# Autodesk Inventor assembly: head
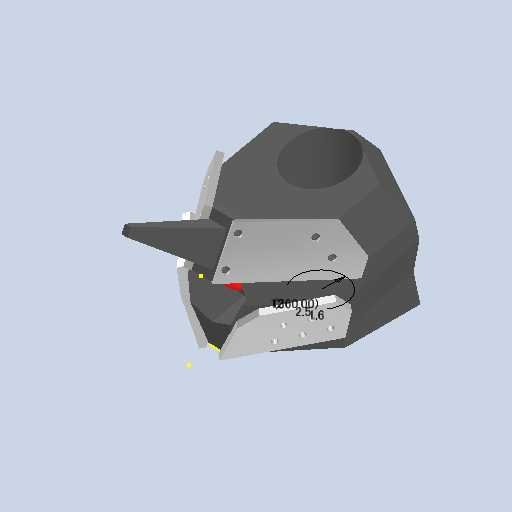
[picture p0: Inventor's stored thumbnail of the model, 512x512]
Saved by Autodesk Inventor 2024.1 (Build 281209000, 209)
## iProperties
Created: 2024-02-25
Part Number: head
Document SubType Name: Assembly
Designer: hibik
Author: hibik
## Documents named in this file (5)
- C:\Users\hibik\Documents\Robomech\HR\Eglantyne\hard\head\head.iam
- C:\Users\hibik\Documents\Robomech\HR\Eglantyne\hard\head\head_bace.ipt
- C:\Users\hibik\Documents\Robomech\HR\Eglantyne\hard\head\face_gard_right.ipt
- C:\Users\hibik\Documents\Robomech\HR\Eglantyne\hard\head\antana.iam
- C:\Users\hibik\Documents\Robomech\HR\Eglantyne\hard\needed_model\KRS3300サーボホーン.ipt
## Components (5 placed, 4 different names)
1. head_bace:1 — メイト:1, メイト:2, メイト:3, メイト:4, メイト:5, メイト:6, メイト:7, メイト:8, メイト:9, メイト:10, 挿入:1, 挿入:2, 挿入:3, 挿入:4
2. face_gard_right:1 — メイト:2, メイト:3, メイト:10, 挿入:1
3. antana:1 [sub-assembly] — メイト:6, メイト:7, 挿入:3
4. face_gard_right:2 — メイト:8, メイト:9, 挿入:2
5. KRS3300サーボホーン:1 — 挿入:4
## Relationships (14: Mate 10, Insert 4)
- メイト:1 [Mate]: head_bace:1
- メイト:2 [Mate]: head_bace:1 ↔ face_gard_right:1
- メイト:3 [Mate]: head_bace:1 ↔ face_gard_right:1
- メイト:4 [Mate]: head_bace:1
- メイト:5 [Mate]: head_bace:1
- メイト:6 [Mate]: head_bace:1 ↔ antana:1
- メイト:7 [Mate]: head_bace:1 ↔ antana:1
- メイト:8 [Mate]: head_bace:1 ↔ face_gard_right:2
- メイト:9 [Mate]: head_bace:1 ↔ face_gard_right:2
- メイト:10 [Mate]: head_bace:1 ↔ face_gard_right:1
- 挿入:1 [Insert]: head_bace:1 ↔ face_gard_right:1
- 挿入:2 [Insert]: head_bace:1 ↔ face_gard_right:2
- 挿入:3 [Insert]: head_bace:1 ↔ antana:1
- 挿入:4 [Insert]: head_bace:1 ↔ KRS3300サーボホーン:1
